# Autodesk Inventor assembly: main_assembly
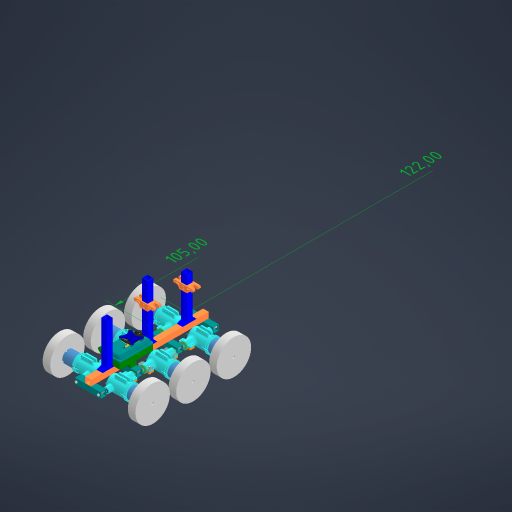
[picture p0: Inventor's stored thumbnail of the model, 512x512]
Saved by Autodesk Inventor 2024 (Build 280153000, 153)
## iProperties
Created: 2023-04-13
Part Number: main_assembly
Document SubType Name: Assembly
Designer: user
Author: user
## Documents named in this file (8)
- D:\Docs\Robot\3d\main_assembly.iam
- D:\Docs\Robot\3d\base\base_assembly.iam
- D:\Docs\Robot\3d\motor_assembly\default_motor_asembly.iam
- D:\Docs\Robot\3d\motor_assembly\holder_assembly.iam
- D:\Docs\Robot\3d\motor_assembly\rigt_motor_asembly.iam
- D:\Docs\Robot\3d\motor_assembly\left_motor_asembly.iam
- D:\Docs\Robot\3d\machine_body\front_box_asembly.iam
- D:\Docs\Robot\3d\machine_body\shock_absorber_holder_up.ipt
## Components (11 placed, 7 different names)
1. base_assembly:1 [sub-assembly] — Совмещение:1, Совмещение:2, Совмещение:3, Совмещение:4, Вставка:1, Совмещение:5, Совмещение:6, Вставка:2, Вставка:3, Вставка:4, Вставка:5, Вставка:6, Совмещение:8, Совмещение:9, Заподлицо:1, Совмещение:10, Совмещение:11, Совмещение:12, Совмещение:13
2. default_motor_asembly:1 [sub-assembly] — Вставка:1, Совмещение:7
3. holder_assembly:1 [sub-assembly] — Совмещение:5, Совмещение:6, Совмещение:7
4. rigt_motor_asembly:1 [sub-assembly] — Вставка:2
5. left_motor_asembly:1 [sub-assembly] — Вставка:3
6. default_motor_asembly:2 [sub-assembly] — Вставка:4
7. rigt_motor_asembly:2 [sub-assembly] — Вставка:5
8. left_motor_asembly:2 [sub-assembly] — Вставка:6
9. front_box_asembly:1 [sub-assembly] — Совмещение:8, Совмещение:9, Заподлицо:1
10. shock_absorber_holder_up:2 — Совмещение:10, Совмещение:11
11. shock_absorber_holder_up:3 — Совмещение:12, Совмещение:13
## Relationships (20: Mate 13, Insert 6, Flush 1)
- Совмещение:1 [Mate]: base_assembly:1
- Совмещение:2 [Mate]: base_assembly:1
- Совмещение:3 [Mate]: base_assembly:1
- Совмещение:4 [Mate]: base_assembly:1
- Вставка:1 [Insert] (11 mm): base_assembly:1 ↔ default_motor_asembly:1
- Совмещение:5 [Mate]: base_assembly:1 ↔ holder_assembly:1
- Совмещение:6 [Mate]: base_assembly:1 ↔ holder_assembly:1
- Совмещение:7 [Mate]: default_motor_asembly:1 ↔ holder_assembly:1
- Вставка:2 [Insert]: base_assembly:1 ↔ rigt_motor_asembly:1
- Вставка:3 [Insert]: base_assembly:1 ↔ left_motor_asembly:1
- Вставка:4 [Insert]: base_assembly:1 ↔ default_motor_asembly:2
- Вставка:5 [Insert]: base_assembly:1 ↔ rigt_motor_asembly:2
- Вставка:6 [Insert]: base_assembly:1 ↔ left_motor_asembly:2
- Совмещение:8 [Mate]: base_assembly:1 ↔ front_box_asembly:1
- Совмещение:9 [Mate]: base_assembly:1 ↔ front_box_asembly:1
- Заподлицо:1 [Flush]: base_assembly:1 ↔ front_box_asembly:1
- Совмещение:10 [Mate]: base_assembly:1 ↔ shock_absorber_holder_up:2
- Совмещение:11 [Mate]: base_assembly:1 ↔ shock_absorber_holder_up:2
- Совмещение:12 [Mate]: base_assembly:1 ↔ shock_absorber_holder_up:3
- Совмещение:13 [Mate]: base_assembly:1 ↔ shock_absorber_holder_up:3
